# Autodesk Inventor assembly: Satellite
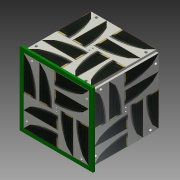
[picture p0: Inventor's stored thumbnail of the model, 180x180]
Saved by Autodesk Inventor 2015 SP1 (Build 190203100, 203)
## iProperties
Created: 2015-06-22
Part Number: Satellite
Document SubType Name: Assembly
Designer: Kartikye
Author: Kartikye
## Documents named in this file (5)
- C:\Users\Kartikye\Documents\GitHub\SASSat\Structure\Satellite.iam
- C:\Users\Kartikye\Documents\GitHub\SASSat\Structure\Corner.ipt
- C:\Users\Kartikye\Documents\GitHub\SASSat\Structure\Solar Panel.iam
- C:\Users\Kartikye\Documents\GitHub\SASSat\Structure\Test Outer Plate.ipt
- C:\Users\Kartikye\Documents\GitHub\SASSat\Structure\Empty Inner PCB.ipt
## Components (16 placed, 4 different names)
1. Corner:1 — Mate:1, Flush:1, Flush:2, Mate:5, Flush:9, Mate:7
2. Corner:2 — Mate:10, Mate:11, Flush:10, Mate:12
3. Corner:3 — Flush:3, Mate:2, Flush:8
4. Corner:4 — Mate:4, Flush:4, Flush:5
5. Corner:5 — Mate:3, Flush:6, Flush:7, Insert:1
6. Solar Panel:1 [sub-assembly] — Mate:1, Flush:1, Flush:2, Flush:3, Mate:2, Mate:3, Mate:4, Flush:4, Flush:5, Flush:6, Flush:7, Flush:8, Mate:6, Mate:8, Mate:25
7. Solar Panel:2 [sub-assembly] — Mate:7, Mate:8, Mate:9, Mate:10, Flush:10, Mate:14, Mate:21
8. Solar Panel:3 [sub-assembly] — Mate:25, Mate:26, Mate:33
9. Solar Panel:4 [sub-assembly] — Mate:18, Mate:19, Mate:26, Mate:28, Mate:29, Mate:36
10. Solar Panel:5 [sub-assembly] — Mate:12, Mate:13, Mate:14, Mate:19, Mate:20, Flush:12, Mate:31, Mate:34
11. Solar Panel:6 [sub-assembly] — Mate:5, Flush:9, Mate:6, Mate:9, Mate:11, Mate:13, Mate:18, Mate:27, Mate:30
12. Corner:6 — Mate:33, Mate:34, Mate:35, Mate:36, Insert:2
13. Corner:7 — Mate:20, Mate:21, Flush:12
14. Corner:8 — Mate:30, Mate:31, Mate:32, Mate:37
15. Test Outer Plate:1 — Mate:27, Mate:28, Mate:29, Mate:32, Mate:35
16. Empty Inner PCB:1 — Mate:37, Insert:1, Insert:2
## Relationships (44: Mate 31, Flush 11, Insert 2)
- Mate:1: Corner:1 ↔ Solar Panel:1
- Flush:1: Corner:1 ↔ Solar Panel:1
- Flush:2: Corner:1 ↔ Solar Panel:1
- Flush:3: Corner:3 ↔ Solar Panel:1
- Mate:2: Corner:3 ↔ Solar Panel:1
- Mate:3: Corner:5 ↔ Solar Panel:1
- Mate:4: Corner:4 ↔ Solar Panel:1
- Flush:4: Corner:4 ↔ Solar Panel:1
- Flush:5: Corner:4 ↔ Solar Panel:1
- Flush:6: Corner:5 ↔ Solar Panel:1
- Flush:7: Corner:5 ↔ Solar Panel:1
- Flush:8: Corner:3 ↔ Solar Panel:1
- Mate:5: Corner:1 ↔ Solar Panel:6
- Flush:9: Corner:1 ↔ Solar Panel:6
- Mate:6: Solar Panel:1 ↔ Solar Panel:6
- Mate:7: Corner:1 ↔ Solar Panel:2
- Mate:8: Solar Panel:1 ↔ Solar Panel:2
- Mate:9: Solar Panel:2 ↔ Solar Panel:6
- Mate:10: Corner:2 ↔ Solar Panel:2
- Mate:11: Corner:2 ↔ Solar Panel:6
- Flush:10: Corner:2 ↔ Solar Panel:2
- Mate:12: Corner:2 ↔ Solar Panel:5
- Mate:13: Solar Panel:5 ↔ Solar Panel:6
- Mate:14: Solar Panel:2 ↔ Solar Panel:5
- Mate:18: Solar Panel:4 ↔ Solar Panel:6
- Mate:19: Solar Panel:4 ↔ Solar Panel:5
- Mate:20: Solar Panel:5 ↔ Corner:7
- Mate:21: Solar Panel:2 ↔ Corner:7
- Flush:12: Solar Panel:5 ↔ Corner:7
- Mate:25: Solar Panel:1 ↔ Solar Panel:3
- Mate:26: Solar Panel:3 ↔ Solar Panel:4
- Mate:27: Solar Panel:6 ↔ Test Outer Plate:1
- Mate:28: Solar Panel:4 ↔ Test Outer Plate:1
- Mate:29: Solar Panel:4 ↔ Test Outer Plate:1
- Mate:30: Solar Panel:6 ↔ Corner:8
- Mate:31: Solar Panel:5 ↔ Corner:8
- Mate:32: Corner:8 ↔ Test Outer Plate:1
- Mate:33: Solar Panel:3 ↔ Corner:6
- Mate:34: Solar Panel:5 ↔ Corner:6
- Mate:35: Corner:6 ↔ Test Outer Plate:1
- Mate:36: Solar Panel:4 ↔ Corner:6
- Mate:37: Corner:8 ↔ Empty Inner PCB:1
- Insert:1: Corner:5 ↔ Empty Inner PCB:1
- Insert:2: Corner:6 ↔ Empty Inner PCB:1
